# Autodesk Inventor assembly: Pull Tester
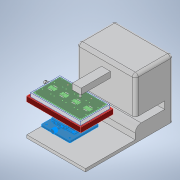
[picture p0: Inventor's stored thumbnail of the model, 180x180]
Saved by Autodesk Inventor 2022 (Build 260153000, 153)
## iProperties
Created: 2020-11-12
Part Number: Pull Tester
Document SubType Name: Assembly
Designer: caleb
Author: caleb
## Documents named in this file (9)
- C:\Users\Caleb\Desktop\nebraska-silicon-lab\Hardware\Pull Tester\Pull Tester.iam
- C:\Users\Caleb\Desktop\nebraska-silicon-lab\Hardware\Pull Tester\Chuck.ipt
- C:\Users\Caleb\Desktop\nebraska-silicon-lab\Hardware\Pull Tester\90128A211_ZNC-PLTD ALLOY STL SCKT HEAD CAP SCREW.ipt
- C:\Users\Caleb\Desktop\nebraska-silicon-lab\Hardware\Pull Tester\step_12694.ipt
- C:\Users\Caleb\Desktop\nebraska-silicon-lab\Hardware\ETL\Module Assembly\Tamale Assembly Plate V2\Tamale Assembly Plate 0p625in with PCB.iam
- C:\Users\Caleb\Desktop\nebraska-silicon-lab\Hardware\Pull Tester\92871A269_18-8 Stainless Steel Unthreaded Spacer.ipt
- C:\Users\Caleb\Desktop\nebraska-silicon-lab\Hardware\Pull Tester\91290A184_Black-Oxide Alloy Steel Socket Head Screw.ipt
- C:\Users\Caleb\Desktop\nebraska-silicon-lab\Hardware\Pull Tester\Royce 610 Base.ipt
- C:\Users\Caleb\Desktop\nebraska-silicon-lab\Hardware\Pull Tester\7397N48_Universal-Thread Push-to-Connect Tube Fittings.ipt
## Components (17 placed, 8 different names)
1. Chuck:1 — Insert:22, Insert:23, Insert:24, Insert:32, Mate:4, Mate:5, Insert:37, Insert:38, Insert:39, Insert:40, Insert:41, Angle:2, Insert:42
2. 90128A211_ZNC-PLTD ALLOY STL SCKT HEAD CAP SCREW:1 — Insert:24, Tangent:3
3. 90128A211_ZNC-PLTD ALLOY STL SCKT HEAD CAP SCREW:2 — Insert:23, Tangent:2
4. 90128A211_ZNC-PLTD ALLOY STL SCKT HEAD CAP SCREW:3 — Insert:22, Tangent:1
5. step_12694:1 — Insert:33, Insert:34, Insert:35, Insert:36, Mate:6, Angle:1, Angle:2
6. 90128A211_ZNC-PLTD ALLOY STL SCKT HEAD CAP SCREW:4 — Insert:32
7. Tamale Assembly Plate 0p625in with PCB:1 [sub-assembly] — Mate:4, Tangent:1, Tangent:2, Tangent:3
8. 92871A269_18-8 Stainless Steel Unthreaded Spacer:1 — Insert:35
9. 92871A269_18-8 Stainless Steel Unthreaded Spacer:2 — Insert:34, Mate:5
10. 92871A269_18-8 Stainless Steel Unthreaded Spacer:3 — Insert:36, Insert:37
11. 92871A269_18-8 Stainless Steel Unthreaded Spacer:4 — Insert:33
12. 91290A184_Black-Oxide Alloy Steel Socket Head Screw:1 — Insert:38
13. 91290A184_Black-Oxide Alloy Steel Socket Head Screw:2 — Insert:39
14. 91290A184_Black-Oxide Alloy Steel Socket Head Screw:3 — Insert:40
15. 91290A184_Black-Oxide Alloy Steel Socket Head Screw:4 — Insert:41
16. Royce 610 Base:1 — Mate:6, Angle:1, Angle:3
17. 7397N48_Universal-Thread Push-to-Connect Tube Fittings:1 — Insert:42, Angle:3
## Relationships (23: Insert 14, Mate 3, Angle 3, Tangent 3)
- Insert:22: Chuck:1 ↔ 90128A211_ZNC-PLTD ALLOY STL SCKT HEAD CAP SCREW:3
- Insert:23: Chuck:1 ↔ 90128A211_ZNC-PLTD ALLOY STL SCKT HEAD CAP SCREW:2
- Insert:24: Chuck:1 ↔ 90128A211_ZNC-PLTD ALLOY STL SCKT HEAD CAP SCREW:1
- Insert:32: Chuck:1 ↔ 90128A211_ZNC-PLTD ALLOY STL SCKT HEAD CAP SCREW:4
- Mate:4: Chuck:1 ↔ Tamale Assembly Plate 0p625in with PCB:1
- Insert:33: step_12694:1 ↔ 92871A269_18-8 Stainless Steel Unthreaded Spacer:4
- Insert:34: step_12694:1 ↔ 92871A269_18-8 Stainless Steel Unthreaded Spacer:2
- Insert:35: step_12694:1 ↔ 92871A269_18-8 Stainless Steel Unthreaded Spacer:1
- Insert:36: step_12694:1 ↔ 92871A269_18-8 Stainless Steel Unthreaded Spacer:3
- Mate:5: Chuck:1 ↔ 92871A269_18-8 Stainless Steel Unthreaded Spacer:2
- Insert:37: Chuck:1 ↔ 92871A269_18-8 Stainless Steel Unthreaded Spacer:3
- Insert:38: Chuck:1 ↔ 91290A184_Black-Oxide Alloy Steel Socket Head Screw:1
- Insert:39: Chuck:1 ↔ 91290A184_Black-Oxide Alloy Steel Socket Head Screw:2
- Insert:40: Chuck:1 ↔ 91290A184_Black-Oxide Alloy Steel Socket Head Screw:3
- Insert:41: Chuck:1 ↔ 91290A184_Black-Oxide Alloy Steel Socket Head Screw:4
- Mate:6: step_12694:1 ↔ Royce 610 Base:1
- Angle:1 (0 deg): step_12694:1 ↔ Royce 610 Base:1
- Angle:2 (0 deg): Chuck:1 ↔ step_12694:1
- Tangent:1: 90128A211_ZNC-PLTD ALLOY STL SCKT HEAD CAP SCREW:3 ↔ Tamale Assembly Plate 0p625in with PCB:1
- Tangent:2: 90128A211_ZNC-PLTD ALLOY STL SCKT HEAD CAP SCREW:2 ↔ Tamale Assembly Plate 0p625in with PCB:1
- Tangent:3: 90128A211_ZNC-PLTD ALLOY STL SCKT HEAD CAP SCREW:1 ↔ Tamale Assembly Plate 0p625in with PCB:1
- Insert:42: Chuck:1 ↔ 7397N48_Universal-Thread Push-to-Connect Tube Fittings:1
- Angle:3 (40 deg): Royce 610 Base:1 ↔ 7397N48_Universal-Thread Push-to-Connect Tube Fittings:1
